# Autodesk Inventor assembly: Assembly2
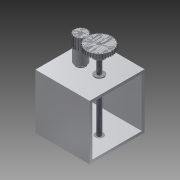
[picture p0: Inventor's stored thumbnail of the model, 180x180]
Saved by Autodesk Inventor 2015 (Build 190159000, 159)
## iProperties
Created: 2015-06-23
Part Number: Assembly2
Document SubType Name: Assembly
Designer: kenta
Author: kenta
## Documents named in this file (8)
- C:\Users\健太\Documents\Inventor\知能ロボコン\Poster presentation\Assembly2.iam
- C:\Users\健太\Documents\Inventor\知能ロボコン\Poster presentation\Square pipe.ipt
- C:\Users\健太\Documents\Inventor\知能ロボコン\Poster presentation\Bearing_MF63ZZ.ipt
- C:\Users\健太\Documents\Inventor\知能ロボコン\Poster presentation\Stopper.ipt
- C:\Users\健太\Documents\Inventor\知能ロボコン\Poster presentation\Shaft 65mm.ipt
- C:\Users\健太\Documents\Inventor\知能ロボコン\Poster presentation\S50D 18K－0803.ipt
- C:\Users\健太\Documents\Inventor\知能ロボコン\Poster presentation\S50D 36B－0303.ipt
- C:\Users\健太\Documents\Inventor\知能ロボコン\Poster presentation\Assembly2\デザイン アクセラレータ\平歯車1.iam
## Components (12 placed, 7 different names)
1. Square pipe:1 — 挿入:1, 挿入:2, 挿入:3, 挿入:4, メイト:1
2. Bearing_MF63ZZ:1 — 挿入:1
3. Bearing_MF63ZZ:2 — 挿入:2, 挿入:20
4. Bearing_MF63ZZ:3 — 挿入:3, 挿入:9
5. Bearing_MF63ZZ:4 — 挿入:4, 挿入:11
6. Stopper:1 — 挿入:11
7. Stopper:2 — 挿入:9, 挿入:10
8. Shaft 65mm:1 — 挿入:10, 挿入:21
9. S50D 18K－0803:1 — 挿入:20, メイト:2, フラッシュ:1, 挿入:22
10. S50D 36B－0303:1 — 挿入:21, メイト:3, フラッシュ:2
11. 平歯車:1 [sub-assembly] — メイト:2, フラッシュ:1, メイト:3, フラッシュ:2
12. Shaft 65mm:2 — 挿入:22
## Relationships (15: Insert 10, Mate 3, Flush 2)
- 挿入:1 [Insert]: Square pipe:1 ↔ Bearing_MF63ZZ:1
- 挿入:2 [Insert]: Square pipe:1 ↔ Bearing_MF63ZZ:2
- 挿入:3 [Insert]: Square pipe:1 ↔ Bearing_MF63ZZ:3
- 挿入:4 [Insert]: Square pipe:1 ↔ Bearing_MF63ZZ:4
- 挿入:9 [Insert]: Bearing_MF63ZZ:3 ↔ Stopper:2
- 挿入:10 [Insert]: Stopper:2 ↔ Shaft 65mm:1
- 挿入:11 [Insert]: Bearing_MF63ZZ:4 ↔ Stopper:1
- メイト:1 [Mate]: Square pipe:1
- 挿入:20 [Insert] (1 mm): Bearing_MF63ZZ:2 ↔ S50D 18K－0803:1
- 挿入:21 [Insert] (-7.8 mm): Shaft 65mm:1 ↔ S50D 36B－0303:1
- メイト:2 [Mate]: S50D 18K－0803:1 ↔ 平歯車:1
- フラッシュ:1 [Flush]: S50D 18K－0803:1 ↔ 平歯車:1
- メイト:3 [Mate]: S50D 36B－0303:1 ↔ 平歯車:1
- フラッシュ:2 [Flush]: S50D 36B－0303:1 ↔ 平歯車:1
- 挿入:22 [Insert]: S50D 18K－0803:1 ↔ Shaft 65mm:2
